# Autodesk Inventor assembly: Marcus' Assembly
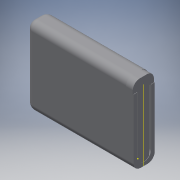
[picture p0: Inventor's stored thumbnail of the model, 180x180]
Saved by Autodesk Inventor 2018 (Build 220112000, 112)
## iProperties
Created: 2019-11-26
Part Number: Marcus' Assembly
Document SubType Name: Assembly
Designer: 871357
Author: 871357
## Documents named in this file (3)
- L:\Marcus' Assembly.iam
- L:\Marcus' Case.ipt
- L:\Marcus' Case Clip.ipt
## Components (2 placed, 2 different names)
1. Marcus' Case:1 — Mate:1, Mate:2
2. Marcus' Case Clip:1 — Mate:1, Mate:2
## Relationships (2: Mate 2)
- Mate:1: Marcus' Case:1 ↔ Marcus' Case Clip:1
- Mate:2 (1.016 mm): Marcus' Case:1 ↔ Marcus' Case Clip:1
